# Autodesk Inventor assembly: TR8_AntiBacklashNut
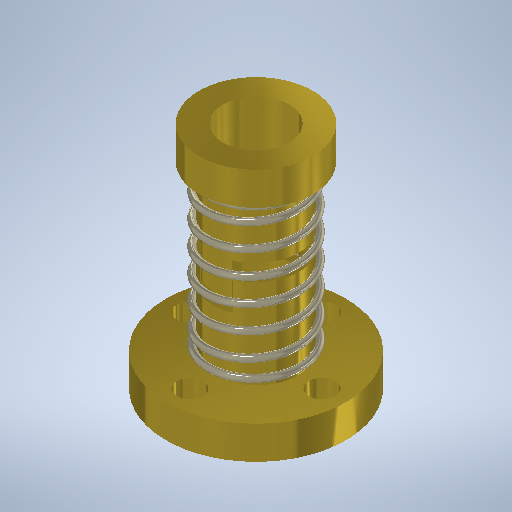
[picture p0: Inventor's stored thumbnail of the model, 512x512]
Saved by Autodesk Inventor 2025.2 (Build 292293000, 293)
## iProperties
Part Number: TR8_AntiBacklashNut
Material: Ogólny
Document SubType Name: Assembly
Designer: user
Author: user
## Documents named in this file (4)
- C:\Users\Simon\OneDrive\Documents\Inventor\Skripsie2025\PartsFolder\Anti-backlash Lead Nut\TR8_AntiBacklashNut.iam
- C:\Users\Simon\OneDrive\Documents\Inventor\Skripsie2025\PartsFolder\Anti-backlash Lead Nut\TR8_AntiBacklashNutMain.ipt
- C:\Users\Simon\OneDrive\Documents\Inventor\Skripsie2025\PartsFolder\Anti-backlash Lead Nut\TR8_AntiBacklashNutSecondary.ipt
- C:\Users\Simon\OneDrive\Documents\Inventor\Skripsie2025\PartsFolder\Anti-backlash Lead Nut\TR8_AntiBacklashNutCoil.ipt
## Components (3 placed, 3 different names)
1. TR8_AntiBacklashNutMain:1 — Zestawiający:2, Zestawiający:3, Równoległy:1, Równoległy:2, Równoległy:3
2. TR8_AntiBacklashNutSecondary:1 — Zestawiający:1, Zestawiający:2, Zestawiający:3, Zestawiający:4
3. TR8_AntiBacklashNutCoil:1 — Zestawiający:1, Zestawiający:4, Równoległy:1, Równoległy:2, Równoległy:3
## Relationships (7: Mate 4, Flush 3)
- Zestawiający:1 [Mate]: TR8_AntiBacklashNutSecondary:1 ↔ TR8_AntiBacklashNutCoil:1
- Zestawiający:2 [Mate]: TR8_AntiBacklashNutMain:1 ↔ TR8_AntiBacklashNutSecondary:1
- Zestawiający:3 [Mate]: TR8_AntiBacklashNutMain:1 ↔ TR8_AntiBacklashNutSecondary:1
- Zestawiający:4 [Mate]: TR8_AntiBacklashNutSecondary:1 ↔ TR8_AntiBacklashNutCoil:1
- Równoległy:1 [Flush]: TR8_AntiBacklashNutMain:1 ↔ TR8_AntiBacklashNutCoil:1
- Równoległy:2 [Flush]: TR8_AntiBacklashNutMain:1 ↔ TR8_AntiBacklashNutCoil:1
- Równoległy:3 [Flush]: TR8_AntiBacklashNutMain:1 ↔ TR8_AntiBacklashNutCoil:1
